# Autodesk Inventor assembly: xy Joiner Left V2 Assembly
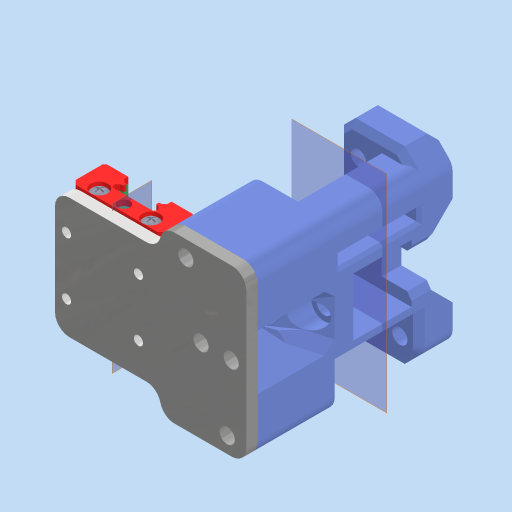
[picture p0: Inventor's stored thumbnail of the model, 512x512]
Saved by Autodesk Inventor 2023.2 (Build 272271000, 271)
## iProperties
Created: 2023-12-06
Part Number: xy Joiner Left V2 Assembly
Document SubType Name: Assembly
Designer: Nils Bade
Author: Nils Bade
## Documents named in this file (4)
- C:\Users\nilsb\Documents\Inventor\Projektarbeit-Bade\RatRig_modified\xy Joiner Left V2 Assembly.iam
- C:\Users\nilsb\Documents\Inventor\Projektarbeit-Bade\RatRig_modified\xy Joiner Left for 4040 V2.ipt
- C:\Users\nilsb\Documents\Inventor\Projektarbeit-Bade\RatRig_modified\XY Joiner Plate for 4040.ipt
- C:\Users\nilsb\Documents\Inventor\Projektarbeit-Bade\RatRig_modified\MGN15 Linear-Rail-Block.ipt
## Components (3 placed, 3 different names)
1. xy Joiner Left for 4040 V2:1 — Passend:1, Passend:2, Passend:3
2. XY Joiner Plate for 4040:1 — Passend:1, Passend:2, Passend:3, Passend:4, Passend:5, Passend:6
3. MGN15 Linear-Rail-Block:1 — Passend:4, Passend:5, Passend:6
## Relationships (6: Mate 6)
- Passend:1 [Mate]: xy Joiner Left for 4040 V2:1 ↔ XY Joiner Plate for 4040:1
- Passend:2 [Mate]: xy Joiner Left for 4040 V2:1 ↔ XY Joiner Plate for 4040:1
- Passend:3 [Mate]: xy Joiner Left for 4040 V2:1 ↔ XY Joiner Plate for 4040:1
- Passend:4 [Mate]: XY Joiner Plate for 4040:1 ↔ MGN15 Linear-Rail-Block:1
- Passend:5 [Mate]: XY Joiner Plate for 4040:1 ↔ MGN15 Linear-Rail-Block:1
- Passend:6 [Mate]: XY Joiner Plate for 4040:1 ↔ MGN15 Linear-Rail-Block:1
